# Autodesk Inventor assembly: ensemble_viseur_amovible
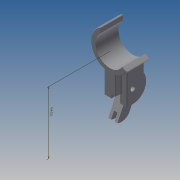
[picture p0: Inventor's stored thumbnail of the model, 180x180]
Saved by Autodesk Inventor 2019 (Build 230136000, 136)
## iProperties
Created: 2019-01-06
Part Number: ensemble_viseur_amovible
Material: Générique
Document SubType Name: Assembly
Designer: Theo
Author: Theo
## Documents named in this file (3)
- D:\dev\projects\canon-ace\ACE 22 A\ensemble_viseur_amovible.iam
- D:\dev\projects\canon-ace\ACE 22 A\viseur_reglable.ipt
- D:\dev\projects\canon-ace\ACE 22 A\viseur_reglable_piece.ipt
## Components (2 placed, 2 different names)
1. viseur_reglable:1 — Placage:2, Placage:3
2. viseur_reglable_piece:1 — Placage:2, Tangente:1, Placage:3
## Relationships (4: Mate 2, Angle 1, Tangent 1)
- Placage:2 [Mate]: viseur_reglable:1 ↔ viseur_reglable_piece:1
- Angle:1 (0 deg)
- Tangente:1: viseur_reglable_piece:1
- Placage:3 [Mate]: viseur_reglable:1 ↔ viseur_reglable_piece:1
